# Autodesk Inventor assembly: A_U_Boot
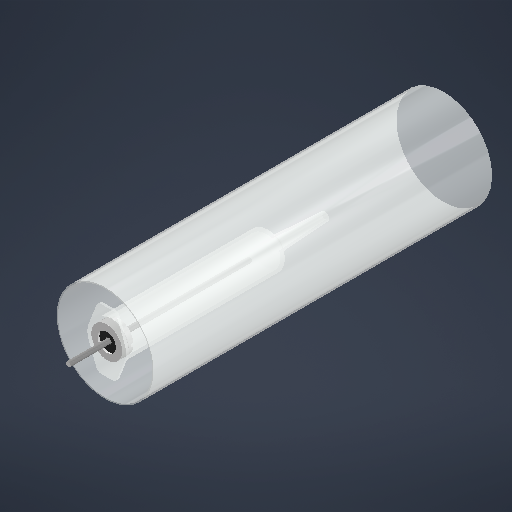
[picture p0: Inventor's stored thumbnail of the model, 512x512]
Saved by Autodesk Inventor 2026 (Build 300175000, 175)
## iProperties
Created: 2025-04-26
Part Number: A_U_Boot
Document SubType Name: Assembly
Designer: FAL
Author: FAL
## Documents named in this file (3)
- C:\Users\FAL\Desktop\git\U-BERT\CAD\A_U-Boot\A_U_Boot.iam
- C:\Users\FAL\Desktop\git\U-BERT\CAD\Trockenzelle\A_Trockenzelle.iam
- C:\Users\FAL\Desktop\git\U-BERT\CAD\Kolbentank\A_Kolbentank.iam
## Components (2 placed, 2 different names)
1. A_Trockenzelle:1 [sub-assembly] — Fluchtend:1, Passend:1, Passend:2
2. A_Kolbentank:1 [sub-assembly] — Fluchtend:2, Passend:3
## Relationships (5: Mate 3, Flush 2)
- Fluchtend:1 [Flush]: A_Trockenzelle:1
- Passend:1 [Mate]: A_Trockenzelle:1
- Passend:2 [Mate]: A_Trockenzelle:1
- Fluchtend:2 [Flush]: A_Kolbentank:1
- Passend:3 [Mate]: A_Kolbentank:1
